# Autodesk Inventor assembly: AxisY
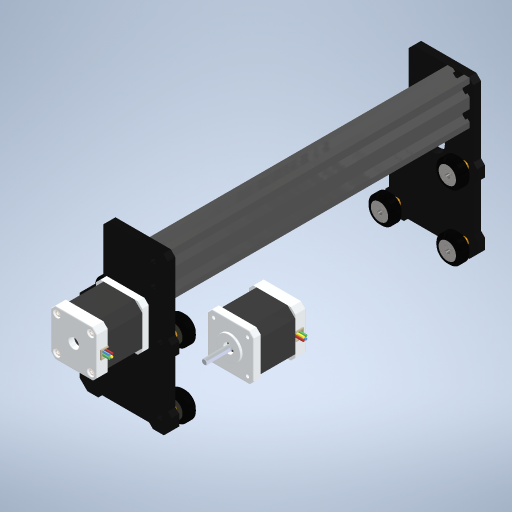
[picture p0: Inventor's stored thumbnail of the model, 512x512]
Saved by Autodesk Inventor 2024.2 (Build 282272000, 272)
## iProperties
Created: 2024-08-27
Part Number: AxisY
Document SubType Name: Assembly
Designer: Admin
Author: Admin
## Documents named in this file (6)
- C:\Users\Admin\Documents\GitHub\RobotCartesiano\DiseñoBrazo\Assemblies\AxisY.iam
- C:\Users\Admin\Documents\GitHub\RobotCartesiano\DiseñoBrazo\Axis\AxisY\AP-Y.ipt
- C:\Users\Admin\Documents\GitHub\RobotCartesiano\DiseñoBrazo\AcrylicPieces\AxisY-Carrier.ipt
- C:\Users\Admin\Documents\GitHub\RobotCartesiano\DiseñoBrazo\AuxiliarPieces\Bearings\625ZZ\NylonPulleyBearing.iam
- C:\Users\Admin\Documents\GitHub\RobotCartesiano\DiseñoBrazo\AuxiliarPieces\M5x6-Insert\M5x6-Insert.ipt
- C:\Users\Admin\Documents\GitHub\RobotCartesiano\DiseñoBrazo\Motors\NEMA17 [48mm]\NEMA17 [48mm].ipt
## Components (21 placed, 5 different names)
1. AP-Y:1 — Mate:1, Mate:2, Mate:3, Mate:4, Mate:5, Mate:6
2. AxisY-Carrier:1 — Mate:1, Mate:2, Mate:3, Mate:15, Mate:16, Mate:17, Mate:18, Mate:19, Mate:20, Mate:21, Mate:22, Mate:39, Mate:40, Mate:41, Mate:42
3. AxisY-Carrier:2 — Mate:4, Mate:5, Mate:6, Mate:31, Mate:32, Mate:33, Mate:34, Mate:35, Mate:36, Mate:37, Mate:38
4. NEMA17 [48mm]:1 — Mate:39, Mate:40, Mate:41, Mate:42
5. NEMA17 [48mm]:3
6. NylonPulleyBearing:9 [sub-assembly] — Mate:7, Mate:8
7. M5x6-Insert:1 — Mate:7, Mate:8, Mate:15, Mate:16
8. NylonPulleyBearing:10 [sub-assembly]
9. M5x6-Insert:2 — Mate:17, Mate:18
10. NylonPulleyBearing:11 [sub-assembly]
11. M5x6-Insert:3 — Mate:21, Mate:22
12. NylonPulleyBearing:12 [sub-assembly]
13. M5x6-Insert:4 — Mate:19, Mate:20
14. M5x6-Insert:6 — Mate:23, Mate:24, Mate:37, Mate:38
15. NylonPulleyBearing:16 [sub-assembly] — Mate:23, Mate:24
16. M5x6-Insert:7 — Mate:31, Mate:32
17. NylonPulleyBearing:17 [sub-assembly]
18. M5x6-Insert:8 — Mate:35, Mate:36
19. NylonPulleyBearing:18 [sub-assembly]
20. M5x6-Insert:9 — Mate:34
21. NylonPulleyBearing:19 [sub-assembly] — Mate:33
## Relationships (42: Mate 42)
- Mate:1: AP-Y:1 ↔ AxisY-Carrier:1
- Mate:2: AP-Y:1 ↔ AxisY-Carrier:1
- Mate:3: AP-Y:1 ↔ AxisY-Carrier:1
- Mate:4: AP-Y:1 ↔ AxisY-Carrier:2
- Mate:5: AP-Y:1 ↔ AxisY-Carrier:2
- Mate:6: AP-Y:1 ↔ AxisY-Carrier:2
- Mate:7: NylonPulleyBearing:9 ↔ M5x6-Insert:1
- Mate:8: NylonPulleyBearing:9 ↔ M5x6-Insert:1
- [Mate]: NylonPulleyBearing:10 ↔ M5x6-Insert:2
- [Mate]: NylonPulleyBearing:10 ↔ M5x6-Insert:2
- [Mate]: NylonPulleyBearing:11 ↔ M5x6-Insert:3
- [Mate]: NylonPulleyBearing:11 ↔ M5x6-Insert:3
- [Mate]: NylonPulleyBearing:12 ↔ M5x6-Insert:4
- [Mate]: NylonPulleyBearing:12 ↔ M5x6-Insert:4
- Mate:15: AxisY-Carrier:1 ↔ M5x6-Insert:1
- Mate:16: AxisY-Carrier:1 ↔ M5x6-Insert:1
- Mate:17: AxisY-Carrier:1 ↔ M5x6-Insert:2
- Mate:18: AxisY-Carrier:1 ↔ M5x6-Insert:2
- Mate:19: AxisY-Carrier:1 ↔ M5x6-Insert:4
- Mate:20: AxisY-Carrier:1 ↔ M5x6-Insert:4
- Mate:21: AxisY-Carrier:1 ↔ M5x6-Insert:3
- Mate:22: AxisY-Carrier:1 ↔ M5x6-Insert:3
- Mate:23: M5x6-Insert:6 ↔ NylonPulleyBearing:16
- Mate:24: M5x6-Insert:6 ↔ NylonPulleyBearing:16
- [Mate]: M5x6-Insert:7 ↔ NylonPulleyBearing:17
- [Mate]: M5x6-Insert:7 ↔ NylonPulleyBearing:17
- [Mate]: M5x6-Insert:8 ↔ NylonPulleyBearing:18
- [Mate]: M5x6-Insert:8 ↔ NylonPulleyBearing:18
- [Mate]: M5x6-Insert:9 ↔ NylonPulleyBearing:19
- [Mate]: M5x6-Insert:9 ↔ NylonPulleyBearing:19
- Mate:31: AxisY-Carrier:2 ↔ M5x6-Insert:7
- Mate:32: AxisY-Carrier:2 ↔ M5x6-Insert:7
- Mate:33: AxisY-Carrier:2 ↔ NylonPulleyBearing:19
- Mate:34: AxisY-Carrier:2 ↔ M5x6-Insert:9
- Mate:35: AxisY-Carrier:2 ↔ M5x6-Insert:8
- Mate:36: AxisY-Carrier:2 ↔ M5x6-Insert:8
- Mate:37: AxisY-Carrier:2 ↔ M5x6-Insert:6
- Mate:38: AxisY-Carrier:2 ↔ M5x6-Insert:6
- Mate:39: AxisY-Carrier:1 ↔ NEMA17 [48mm]:1
- Mate:40: AxisY-Carrier:1 ↔ NEMA17 [48mm]:1
- Mate:41: AxisY-Carrier:1 ↔ NEMA17 [48mm]:1
- Mate:42: AxisY-Carrier:1 ↔ NEMA17 [48mm]:1
## Named parameters: d8_d6 = 0 mm, d9_d7 = 0 mm, d10_d6 = 0 mm, d11_d7 = 0 mm, d12_d6 = 0 mm, d13_d7 = 0 mm, d24_d22 = 0 mm, d25_d23 = 0 mm, d26_d22 = 0 mm, d27_d23 = 0 mm, d28_d22 = 0 mm, d29_d23 = 0 mm
